# Autodesk Inventor assembly: Gripper Assembly
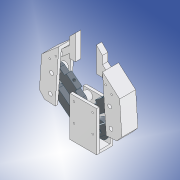
[picture p0: Inventor's stored thumbnail of the model, 180x180]
Saved by Autodesk Inventor 2017 (Build 210142000, 142)
## iProperties
Created: 2017-06-19
Part Number: Gripper Assembly
Document SubType Name: Assembly
Designer: Zach
Author: Zach
## Documents named in this file (8)
- C:\Users\zallen\Documents\GitHub\cr-laundry-robot\src\Body\Arm Assembly\Gripper Assembly\Gripper Assembly.iam
- C:\Users\zallen\Documents\GitHub\cr-laundry-robot\src\Body\Arm Assembly\Gripper Assembly\GA001.ipt
- C:\Users\zallen\Documents\GitHub\cr-laundry-robot\src\Body\Arm Assembly\Gripper Assembly\GA002.ipt
- C:\Users\zallen\Documents\GitHub\cr-laundry-robot\src\Body\Arm Assembly\Gripper Assembly\GA003.ipt
- C:\Users\zallen\Documents\GitHub\cr-laundry-robot\src\Body\Arm Assembly\Gripper Assembly\GA004.ipt
- C:\Users\zallen\Documents\GitHub\cr-laundry-robot\src\Body\Arm Assembly\Gripper Assembly\GA005.ipt
- C:\Users\zallen\Documents\GitHub\cr-laundry-robot\src\Body\Arm Assembly\Gripper Assembly\GA006.ipt
- C:\Users\zallen\Documents\GitHub\cr-laundry-robot\src\Body\Arm Assembly\Gripper Assembly\GA007.ipt
## Components (12 placed, 7 different names)
1. GA001:1 — Mate:1, Mate:3, Mate:4, Mate:5, Mate:7, Mate:9, Mate:12, Mate:16, Mate:20, Mate:21, Mate:22, Mate:33, Mate:38, Mate:39, Mate:40
2. GA002:1 — Mate:1, Mate:10, Mate:11, Mate:33
3. GA002:2 — Mate:3, Mate:4, Mate:13, Mate:14
4. GA003:1 — Mate:5, Mate:16, Mate:18
5. GA003:2 — Mate:7, Mate:23, Mate:41
6. GA004:1 — Mate:9, Mate:10, Mate:11, Mate:17, Mate:34, Symmetry:1
7. GA004:2 — Mate:12, Mate:13, Mate:14, Mate:24, Mate:35, Symmetry:1
8. GA005:1 — Mate:17, Mate:18, Mate:29, Mate:30, Mate:34, Mate:37, Symmetry:2
9. GA005:2 — Mate:23, Mate:24, Mate:26, Mate:27, Mate:35, Mate:36, Mate:41, Symmetry:2
10. GA006:1 — Mate:20, Mate:21, Mate:22
11. GA007:1 — Mate:26, Mate:27, Mate:36
12. GA007:2 — Mate:29, Mate:30, Mate:37
## Relationships (34: Mate 32, Symmetry 2)
- Mate:1: GA001:1 ↔ GA002:1
- Mate:3: GA001:1 ↔ GA002:2
- Mate:4: GA001:1 ↔ GA002:2
- Mate:5: GA001:1 ↔ GA003:1
- Mate:7: GA001:1 ↔ GA003:2
- Mate:9: GA001:1 ↔ GA004:1
- Mate:10: GA002:1 ↔ GA004:1
- Mate:11: GA002:1 ↔ GA004:1
- Mate:12: GA001:1 ↔ GA004:2
- Mate:13: GA002:2 ↔ GA004:2
- Mate:14: GA002:2 ↔ GA004:2
- Mate:16: GA001:1 ↔ GA003:1
- Mate:17: GA004:1 ↔ GA005:1
- Mate:18: GA003:1 ↔ GA005:1
- Mate:20: GA001:1 ↔ GA006:1
- Mate:21: GA001:1 ↔ GA006:1
- Mate:22: GA001:1 ↔ GA006:1
- Mate:23: GA003:2 ↔ GA005:2
- Mate:24: GA004:2 ↔ GA005:2
- Mate:26: GA005:2 ↔ GA007:1
- Mate:27: GA005:2 ↔ GA007:1
- Mate:29: GA005:1 ↔ GA007:2
- Mate:30: GA005:1 ↔ GA007:2
- Mate:33: GA001:1 ↔ GA002:1
- Mate:34: GA004:1 ↔ GA005:1
- Mate:35: GA004:2 ↔ GA005:2
- Mate:36: GA005:2 ↔ GA007:1
- Mate:37: GA005:1 ↔ GA007:2
- Mate:38: GA001:1
- Mate:39: GA001:1
- Mate:40: GA001:1
- Symmetry:1: GA004:1 ↔ GA004:2
- Mate:41: GA003:2 ↔ GA005:2
- Symmetry:2: GA005:1 ↔ GA005:2
